# Autodesk Inventor assembly: lemon shape asse
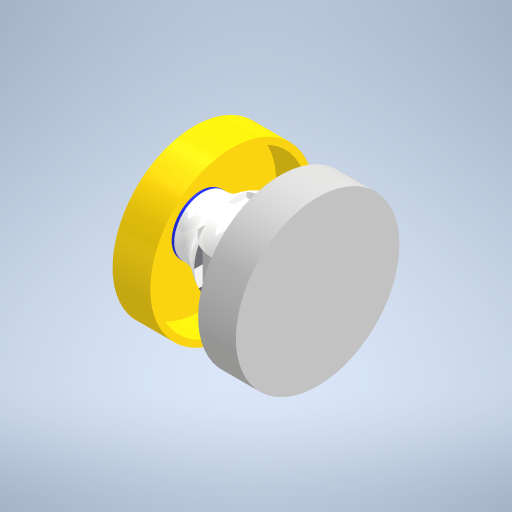
[picture p0: Inventor's stored thumbnail of the model, 512x512]
Saved by Autodesk Inventor 2023 (Build 270158000, 158)
## iProperties
Created: 2022-11-14
Part Number: lemon shape asse
Document SubType Name: Assembly
Designer: RM206user
Author: RM206user
## Documents named in this file (10)
- C:\Users\RM206user\Desktop\cansat\tanekonsat2022_runback\machinary\parts\tire\lemon shape asse.iam
- C:\Users\RM206user\Desktop\cansat\tanekonsat2022_runback\machinary\parts\bush.ipt
- C:\Users\RM206user\Desktop\cansat\tanekonsat2022_runback\machinary\body\body back\back moter middle tire ver\back moter middle tire lemon shape.ipt
- C:\Users\RM206user\Desktop\cansat\tanekonsat2022_runback\machinary\body\body front\front moter middle basic\body front moter middle lemon shape.ipt
- C:\Users\RM206user\Desktop\cansat\tanekonsat2022_runback\machinary\body\body back\back for main connection\body back for main 3.ipt
- C:\Users\RM206user\Desktop\cansat\tanekonsat2022_runback\machinary\parts\GNSS1.ipt
- C:\Users\RM206user\Desktop\cansat\tanekonsat2022_runback\machinary\parts\almi1.ipt
- C:\Users\RM206user\Desktop\cansat\tanekonsat2022_runback\machinary\parts\almi2.ipt
- C:\Users\RM206user\Desktop\cansat\tanekonsat2022_runback\machinary\parts\mein1.ipt
- C:\Users\RM206user\Desktop\cansat\tanekonsat2022_runback\machinary\parts\tire\tire out130 in 22 5mm inward.ipt
## Components (11 placed, 9 different names)
1. bush:1 — メイト:37, メイト:38, メイト:43, メイト:44
2. bush:2 — メイト:39, メイト:40, メイト:41, メイト:42
3. body moter middle:1 — メイト:1, メイト:2, メイト:26, メイト:31, メイト:32, メイト:33, メイト:34, メイト:35, メイト:36
4. base front:1 — メイト:3, メイト:4, メイト:5, メイト:6, メイト:7, メイト:8, メイト:9, メイト:13, メイト:14, メイト:15, メイト:16, メイト:17, メイト:34, メイト:35, メイト:36, メイト:37, メイト:38, メイト:39, メイト:40
5. body back:1 — メイト:1, メイト:2, メイト:26
6. GNSS1:1 — メイト:13, メイト:14, メイト:15
7. almi1:1 — メイト:6, メイト:7, メイト:16
8. almi2:1 — メイト:3, メイト:4, メイト:5
9. mein1:1 — メイト:8, メイト:9, メイト:17
10. tire out130 in 22 5mm inward:1 — メイト:43, メイト:44
11. tire out130 in 22 5mm inward:2 — メイト:41, メイト:42
## Relationships (29: Mate 29)
- メイト:1 [Mate]: body moter middle:1 ↔ body back:1
- メイト:2 [Mate]: body moter middle:1 ↔ body back:1
- メイト:3 [Mate]: base front:1 ↔ almi2:1
- メイト:4 [Mate]: base front:1 ↔ almi2:1
- メイト:5 [Mate]: base front:1 ↔ almi2:1
- メイト:6 [Mate]: base front:1 ↔ almi1:1
- メイト:7 [Mate]: base front:1 ↔ almi1:1
- メイト:8 [Mate]: base front:1 ↔ mein1:1
- メイト:9 [Mate]: base front:1 ↔ mein1:1
- メイト:13 [Mate]: base front:1 ↔ GNSS1:1
- メイト:14 [Mate]: base front:1 ↔ GNSS1:1
- メイト:15 [Mate]: base front:1 ↔ GNSS1:1
- メイト:16 [Mate]: base front:1 ↔ almi1:1
- メイト:17 [Mate]: base front:1 ↔ mein1:1
- メイト:26 [Mate]: body moter middle:1 ↔ body back:1
- メイト:31 [Mate]: body moter middle:1
- メイト:32 [Mate]: body moter middle:1
- メイト:33 [Mate]: body moter middle:1
- メイト:34 [Mate]: body moter middle:1 ↔ base front:1
- メイト:35 [Mate]: body moter middle:1 ↔ base front:1
- メイト:36 [Mate]: body moter middle:1 ↔ base front:1
- メイト:37 [Mate]: bush:1 ↔ base front:1
- メイト:38 [Mate]: bush:1 ↔ base front:1
- メイト:39 [Mate]: bush:2 ↔ base front:1
- メイト:40 [Mate]: bush:2 ↔ base front:1
- メイト:41 [Mate]: bush:2 ↔ tire out130 in 22 5mm inward:2
- メイト:42 [Mate]: bush:2 ↔ tire out130 in 22 5mm inward:2
- メイト:43 [Mate]: bush:1 ↔ tire out130 in 22 5mm inward:1
- メイト:44 [Mate]: bush:1 ↔ tire out130 in 22 5mm inward:1
